# Autodesk Inventor assembly: FE-00036LowerFrame
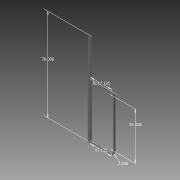
[picture p0: Inventor's stored thumbnail of the model, 180x180]
Saved by Autodesk Inventor 2013 (Build 170138000, 138)
## iProperties
Created: 2013-01-13
Part Number: FE-00036LowerFrame
Document SubType Name: Assembly
Designer: Phillip
Author: Phillip
## Documents named in this file (5)
- C:\Users\Moses\Documents\Inventor\2013 Team 3061 Robot\FIRST Arena 2013\Feeder Goal Station\FE-00036LowerFrame.iam
- C:\Users\Moses\Documents\Inventor\2013 Team 3061 Robot\FIRST Arena 2013\Feeder Goal Station\FE00036LowerFrame.ipt
- C:\Users\Moses\Documents\Inventor\2013 Team 3061 Robot\FIRST Arena 2013\Feeder Goal Station\FE-00036LowerFrame\Frame\Frame0001.iam
- C:\Users\Moses\Documents\Inventor\2013 Team 3061 Robot\FIRST Arena 2013\Feeder Goal Station\Frame0002.ipt
- C:\Users\Moses\Documents\Inventor\2013 Team 3061 Robot\FIRST Arena 2013\Feeder Goal Station\FE-00036Base.ipt
## Components (4 placed, 4 different names)
1. FE00036LowerFrame:1
2. Frame0001:1 [sub-assembly] — Mate:1
3. Frame0002:1 — Flush:1, Flush:2
4. FE-00036Base:1 — Flush:2
## Relationships (3: Flush 2, Mate 1)
- Flush:1: Frame0002:1
- Flush:2: Frame0002:1 ↔ FE-00036Base:1
- Mate:1: Frame0001:1
